# Autodesk Inventor assembly: photodetector_assembly
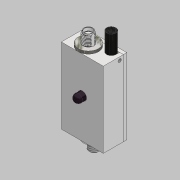
[picture p0: Inventor's stored thumbnail of the model, 180x180]
Saved by Autodesk Inventor 2021.4 (Build 254397000, 397)
## iProperties
Created: 2022-11-02
Part Number: photodetector_assembly
Document SubType Name: Assembly
Designer: Tilman Preuschoff
Author: Tilman Preuschoff
## Documents named in this file (8)
- C:\Users\Tilman Preuschoff\Documents\GitHub\SFH203_photodetector\case\assembly\photodetector_assembly.iam
- C:\Users\Tilman Preuschoff\Documents\GitHub\SFH203_photodetector\case\case.ipt
- C:\Users\Tilman Preuschoff\Documents\GitHub\SFH203_photodetector\case\assembly\SFH203_photodetector.iam
- C:\Users\Tilman Preuschoff\Documents\Inventor\Content Center Files\R2021\de-DE\DIN 84\DIN 84 - M2,5 x 5.ipt
- C:\Users\Tilman Preuschoff\Documents\Inventor\Content Center Files\R2021\de-DE\DIN 125-1  A\DIN 125 - A 6,4.ipt
- C:\Users\Tilman Preuschoff\Documents\Inventor\Content Center Files\R2021\de-DE\DIN 914\DIN 914 - M6 x 16.ipt
- C:\Users\Tilman Preuschoff\Documents\GitHub\SFH203_photodetector\case\cover.ipt
- C:\Users\Tilman Preuschoff\Documents\GitHub\SFH203_photodetector\case\assembly\cable.ipt
## Components (10 placed, 7 different names)
1. case:1 — Passend:1, Passend:3, Winkel:1, Drehbar:5, Starr:1, Passend:5, Passend:7, Winkel:3, Passend:11, Passend:12, Passend:13, Winkel:4, Winkel:5, Tangential:1, Tangential:2, Passend:14
2. DIN 84 - ersetzt durch DIN EN ISO 1207 M2,5 x 5:3
3. DIN 84 - ersetzt durch DIN EN ISO 1207 M2,5 x 5:4
4. DIN 125-1 A A 6,4:1 — Starr:1
5. DIN 914 M6 x 16:1 — Drehbar:5
6. DIN 125-1 A A 6,4:2 — Passend:5
7. cover:1 — Passend:7, Winkel:3, Passend:14
8. SFH203_photodetector:1 [sub-assembly] — Passend:12, Passend:13, Winkel:4
9. DIN 125-1 A A 6,4:3 — Passend:11
10. cable:1 — Winkel:5, Tangential:1, Tangential:2
## Relationships (16: Mate 8, Angle 4, Tangent 2, RevoluteJoint 1, WeldJoint 1)
- Passend:1 [Mate]: case:1
- Passend:3 [Mate]: case:1
- Winkel:1 [Angle] (0 deg): case:1
- Drehbar:5 [RevoluteJoint] (6 mm): case:1 ↔ DIN 914 M6 x 16:1
- Starr:1 [WeldJoint]: case:1 ↔ DIN 125-1 A A 6,4:1
- Passend:5 [Mate]: case:1 ↔ DIN 125-1 A A 6,4:2
- Passend:7 [Mate]: case:1 ↔ cover:1
- Winkel:3 [Angle] (180 deg): case:1 ↔ cover:1
- Passend:11 [Mate]: case:1 ↔ DIN 125-1 A A 6,4:3
- Passend:12 [Mate]: case:1 ↔ SFH203_photodetector:1
- Passend:13 [Mate]: case:1 ↔ SFH203_photodetector:1
- Winkel:4 [Angle] (0 deg): case:1 ↔ SFH203_photodetector:1
- Winkel:5 [Angle] (0 deg): case:1 ↔ cable:1
- Tangential:1: case:1 ↔ cable:1
- Tangential:2: case:1 ↔ cable:1
- Passend:14 [Mate]: case:1 ↔ cover:1
